# Autodesk Inventor assembly: A2017_T2_00
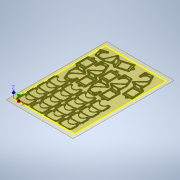
[picture p0: Inventor's stored thumbnail of the model, 180x180]
Saved by Autodesk Inventor 2020 (Build 240168000, 168)
## iProperties
Created: 2021-08-27
Part Number: A2017_T2_00
Document SubType Name: Assembly
Designer: Masato
Author: Masato
## Documents named in this file (4)
- D:\GitHub\inventor\SUSTAINA-OP\Cam\A2017_T2_11.iam
- D:\GitHub\inventor\SUSTAINA-OP\Cam\DisposableBoard.ipt
- D:\GitHub\inventor\SUSTAINA-OP\LowerBody\Ankle\Ankle_side_frame.ipt
- D:\GitHub\inventor\SUSTAINA-OP\LowerBody\Ankle\Ankle_back_frame.ipt
## Components (23 placed, 3 different names)
1. DisposableBoard:1 — メイト:2, メイト:1, フラッシュ:1, フラッシュ:2, メイト:10, メイト:11, メイト:12, メイト:14, メイト:15, メイト:17, メイト:19, メイト:20, 正接:1, 正接:2, 正接:6
2. Ankle_side_frame:10 — メイト:20, 正接:4, 正接:5, 正接:6
3. Ankle_side_frame:11 — メイト:19, 正接:1, 正接:2, 正接:3
4. Ankle_back_frame:16 — メイト:10, メイト:11, メイト:12
5. Ankle_back_frame:17
6. Ankle_back_frame:18
7. Ankle_back_frame:19 — メイト:13
8. Ankle_back_frame:20
9. Ankle_back_frame:21
10. Ankle_back_frame:22
11. Ankle_back_frame:23
12. Ankle_back_frame:24
13. Ankle_back_frame:25
14. Ankle_back_frame:26
15. Ankle_back_frame:27
16. Ankle_back_frame:28
17. Ankle_back_frame:29
18. Ankle_back_frame:30
19. Ankle_back_frame:31
20. Ankle_side_frame:6 — メイト:13, メイト:14, メイト:15, メイト:16, メイト:18
21. Ankle_side_frame:7 — メイト:16, メイト:17, メイト:18, 正接:3
22. Ankle_side_frame:8
23. Ankle_side_frame:9 — 正接:4, 正接:5
## Component patterns: (16 elements, first: Ankle_back_frame:16), (2 elements, first: Ankle_side_frame:6 + Ankle_side_frame:7)
## Relationships (21: Mate 13, Tangent 6, Flush 2)
- メイト:2 [Mate]: DisposableBoard:1
- メイト:1 [Mate]: DisposableBoard:1
- フラッシュ:1 [Flush]: DisposableBoard:1
- フラッシュ:2 [Flush]: DisposableBoard:1
- メイト:10 [Mate]: DisposableBoard:1 ↔ Ankle_back_frame:16
- メイト:11 [Mate] (2 mm): DisposableBoard:1 ↔ Ankle_back_frame:16
- メイト:12 [Mate] (2 mm): DisposableBoard:1 ↔ Ankle_back_frame:16
- メイト:13 [Mate] (2.5 mm): Ankle_back_frame:19 ↔ Ankle_side_frame:6
- メイト:14 [Mate] (2 mm): DisposableBoard:1 ↔ Ankle_side_frame:6
- メイト:15 [Mate]: DisposableBoard:1 ↔ Ankle_side_frame:6
- メイト:16 [Mate] (2.5 mm): Ankle_side_frame:6 ↔ Ankle_side_frame:7
- メイト:17 [Mate]: DisposableBoard:1 ↔ Ankle_side_frame:7
- メイト:18 [Mate] (2.5 mm): Ankle_side_frame:6 ↔ Ankle_side_frame:7
- メイト:19 [Mate]: DisposableBoard:1 ↔ Ankle_side_frame:11
- メイト:20 [Mate]: DisposableBoard:1 ↔ Ankle_side_frame:10
- 正接:1 [Tangent] (5 mm): DisposableBoard:1 ↔ Ankle_side_frame:11
- 正接:2 [Tangent] (2 mm): DisposableBoard:1 ↔ Ankle_side_frame:11
- 正接:3 [Tangent] (2.5 mm): Ankle_side_frame:11 ↔ Ankle_side_frame:7
- 正接:4 [Tangent] (2.5 mm): Ankle_side_frame:10 ↔ Ankle_side_frame:9
- 正接:5 [Tangent] (2.5 mm): Ankle_side_frame:10 ↔ Ankle_side_frame:9
- 正接:6 [Tangent] (4 mm): DisposableBoard:1 ↔ Ankle_side_frame:10
